# Autodesk Inventor assembly: ヘッケン＋揺動節1_MIR
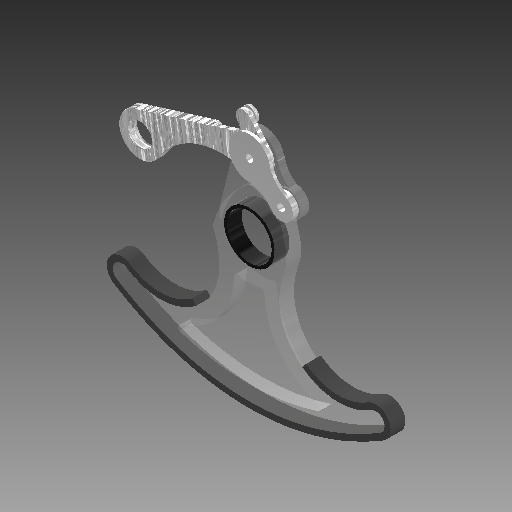
[picture p0: Inventor's stored thumbnail of the model, 512x512]
Saved by Autodesk Inventor 2020 (Build 240168000, 168)
## iProperties
Created: 2019-07-24
Part Number: ヘッケン＋揺動節1_MIR
Document SubType Name: Assembly
Designer: 雪村
Mass: 14.4445 g
Surface Area: 117.972 cm^2
Volume: 10.3899 cm^3
Density: 1.39025 g/cm^3
Author: 雪村
## Documents named in this file (7)
- C:\Users\white\Documents\SRDC\SRDC\Inventor_2017\2018年機体\2020年4年機体\ヘッケン＋揺動節1_MIR.iam
- C:\Users\white\Documents\SRDC\SRDC\Inventor_2017\2018年機体\2020年4年機体\ヘッケン1_MIR.ipt
- C:\Users\white\Documents\SRDC\SRDC\Inventor_2017\2018年機体\2020年4年機体\脚揺動節1_MIR.ipt
- C:\Users\white\Documents\SRDC\SRDC\Inventor_2017\2018年機体\パーツ\オイレス060801.5.ipt
- C:\Users\white\Documents\SRDC\SRDC\Inventor_2017\2018年機体\2020年4年機体\脚揺動節抑え1.ipt
- C:\Users\white\Documents\SRDC\SRDC\Inventor_2017\2018年機体\パーツ\オイレス151705.ipt
- C:\Users\white\Documents\SRDC\SRDC\Inventor_2017\2018年機体\2020年4年機体\脚ゴム1.ipt
## Components (6 placed, 6 different names)
1. ヘッケン1_MIR:1
2. 脚揺動節1_MIR:1
3. オイレス060801.5:1
4. 脚揺動節抑え1:1
5. オイレス151705:1
6. 脚ゴム1:1
## Relationships (7: Insert 7)
- [Insert]: 脚揺動節1_MIR:1 ↔ オイレス060801.5:1
- [Insert]: ヘッケン1_MIR:1 ↔ オイレス060801.5:1
- [Insert]: ヘッケン1_MIR:1 ↔ 脚揺動節抑え1:1
- [Insert]: ヘッケン1_MIR:1 ↔ 脚揺動節抑え1:1
- [Insert]: ヘッケン1_MIR:1 ↔ オイレス151705:1
- [Insert]: ヘッケン1_MIR:1 ↔ 脚ゴム1:1
- [Insert]: ヘッケン1_MIR:1 ↔ 脚ゴム1:1
